# Autodesk Inventor assembly: Base Chassis Assembly
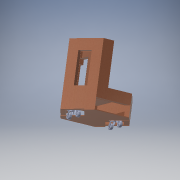
[picture p0: Inventor's stored thumbnail of the model, 180x180]
Saved by Autodesk Inventor 2017 (Build 210142000, 142)
## iProperties
Created: 2018-10-18
Part Number: Base Chassis Assembly
Document SubType Name: Assembly
Designer: Dell
Author: Dell
## Documents named in this file (13)
- C:\Users\Dell\Documents\GitHub\tr2\Base\Base Chassis Assembly.iam
- C:\Users\Dell\Documents\GitHub\tr2\BA01.ipt
- C:\Users\Dell\Documents\GitHub\tr2\BA02.ipt
- C:\Users\Dell\Documents\GitHub\tr2\Base\BA07.ipt
- C:\Users\Dell\Documents\GitHub\tr2\Base\BA08.ipt
- C:\Users\Dell\Documents\GitHub\tr2\Base\BA11.ipt
- C:\Users\Dell\Documents\GitHub\tr2\Base\BA015.ipt
- C:\Users\Dell\Documents\GitHub\tr2\Base\Caster 2in.ipt
- C:\Users\Dell\Documents\GitHub\tr2\Base\BA16.ipt
- C:\Users\Dell\Documents\GitHub\tr2\Base\BA17.ipt
- C:\Users\Dell\Documents\GitHub\tr2\Base\BA18.ipt
- C:\Users\Dell\Documents\GitHub\tr2\Base\BA22.ipt
- C:\Users\Dell\Documents\GitHub\tr2\Base\BA23.ipt
## Components (34 placed, 12 different names)
1. BA01:1
2. BA01:2 — Flush:33
3. BA01:3
4. BA01:4 — Flush:24
5. BA01:5 — Flush:32, Mate:65, Mate:67
6. BA01:6
7. BA01:7 — Mate:45, Flush:25, Mate:60
8. BA01:8 — Mate:47, Flush:26, Mate:49, Mate:55
9. BA01:9 — Mate:46, Mate:48, Mate:50, Mate:56
10. BA01:10 — Flush:24, Mate:45, Flush:25, Mate:61
11. BA02:2 — Mate:66, Mate:67, Flush:33
12. BA02:4 — Mate:64
13. BA02:5 — Flush:32, Mate:64, Mate:65, Mate:66
14. BA07:1
15. BA07:2
16. BA07:3 — Mate:76
17. BA07:4
18. BA07:5 — Mate:69, Mate:75, Flush:37
19. BA07:6 — Mate:71, Mate:74
20. BA08:1
21. BA08:2 — Mate:72
22. BA11:1 — Mate:68, Flush:34
23. BA015:1 — Mate:46, Mate:47, Mate:48
24. BA16:1 — Flush:26, Mate:49, Mate:50, Mate:51, Mate:53, Mate:54, Flush:27, Flush:29
25. BA16:2 — Mate:60, Mate:61, Flush:29, Flush:30, Flush:31
26. BA17:1 — Mate:68, Flush:34, Mate:69, Mate:70, Flush:35, Flush:36, Mate:73, Mate:77
27. BA18:1 — Mate:70, Flush:35, Mate:71
28. BA18:2 — Flush:36, Mate:72, Mate:73, Flush:38
29. Caster 2in:1 — Mate:51, Flush:27, Mate:55, Mate:63
30. Caster 2in:2 — Mate:53, Mate:54, Mate:56, Mate:62
31. Caster 2in:3 — Flush:31, Mate:63
32. Caster 2in:4 — Mate:62, Flush:30
33. BA22:1 — Mate:74, Mate:75, Flush:37
34. BA23:1 — Mate:76, Flush:38, Mate:77
## Relationships (100: Mate 68, Flush 32)
- [Mate]: BA01:1 ↔ BA01:6
- [Mate]: BA01:2 ↔ BA01:6
- [Mate]: BA01:2 ↔ BA01:6
- [Mate]: BA01:2 ↔ BA01:6
- [Flush]: BA01:1 ↔ BA01:6
- [Mate]: BA01:1 ↔ BA01:6
- [Mate]: BA01:2 ↔ BA01:3
- [Mate]: BA01:2 ↔ BA01:3
- [Flush]: BA01:2 ↔ BA01:3
- [Mate]: BA01:1 ↔ BA01:5
- [Flush]: BA01:1 ↔ BA01:5
- [Mate]: BA01:1 ↔ BA01:5
- [Mate]: BA01:4 ↔ BA01:5
- [Flush]: BA01:4 ↔ BA01:5
- [Mate]: BA01:4 ↔ BA01:5
- [Mate]: BA01:3 ↔ BA01:7
- [Mate]: BA01:3 ↔ BA01:7
- [Mate]: BA01:2 ↔ BA01:7
- [Flush]: BA01:6 ↔ BA01:8
- [Mate]: BA01:2 ↔ BA01:8
- [Mate]: BA01:6 ↔ BA01:8
- [Mate]: BA01:6 ↔ BA01:8
- [Mate]: BA01:8 ↔ BA01:9
- [Mate]: BA01:5 ↔ BA01:9
- [Mate]: BA01:1 ↔ BA01:9
- [Mate]: BA01:4 ↔ BA07:1
- [Flush]: BA01:4 ↔ BA07:1
- [Mate]: BA01:4 ↔ BA07:1
- [Mate]: BA07:1 ↔ BA07:2
- [Flush]: BA07:1 ↔ BA07:2
- [Flush]: BA01:3 ↔ BA07:2
- [Mate]: BA01:4 ↔ BA07:3
- [Flush]: BA07:1 ↔ BA07:3
- [Mate]: BA01:5 ↔ BA07:3
- [Mate]: BA07:3 ↔ BA07:4
- [Mate]: BA07:5 ↔ BA07:6
- [Mate]: BA07:5 ↔ BA07:6
- [Flush]: BA07:5 ↔ BA07:6
- [Mate]: BA01:2 ↔ BA07:6
- [Mate]: BA01:3 ↔ BA07:6
- [Flush]: BA01:7 ↔ BA07:6
- [Mate]: BA07:2 ↔ BA08:1
- [Flush]: BA07:2 ↔ BA08:1
- [Flush]: BA07:2 ↔ BA08:1
- [Mate]: BA07:1 ↔ BA08:2
- [Flush]: BA07:1 ↔ BA08:2
- [Flush]: BA07:1 ↔ BA08:2
- [Mate]: BA07:3 ↔ BA07:4
- [Mate]: BA01:5 ↔ BA07:4
- [Flush]: BA02:4 ↔ BA07:5
- [Mate]: BA02:4 ↔ BA07:4
- [Flush] (-44.45 mm): BA01:2 ↔ BA02:4
- [Mate]: BA02:4 ↔ BA11:1
- [Flush]: BA02:4 ↔ BA11:1
- [Mate] (171.45 mm): BA07:4 ↔ BA11:1
- Flush:24: BA01:4 ↔ BA01:10
- Mate:45: BA01:7 ↔ BA01:10
- Flush:25: BA01:7 ↔ BA01:10
- Mate:46: BA01:9 ↔ BA015:1
- Mate:47: BA01:8 ↔ BA015:1
- Mate:48: BA01:9 ↔ BA015:1
- Flush:26 (19.05 mm): BA01:8 ↔ BA16:1
- Mate:49: BA01:8 ↔ BA16:1
- Mate:50: BA01:9 ↔ BA16:1
- Mate:51: BA16:1 ↔ Caster 2in:1
- Mate:53: BA16:1 ↔ Caster 2in:2
- Mate:54: BA16:1 ↔ Caster 2in:2
- Flush:27: BA16:1 ↔ Caster 2in:1
- Mate:55 (12.7 mm): BA01:8 ↔ Caster 2in:1
- Mate:56 (12.7 mm): BA01:9 ↔ Caster 2in:2
- [Mate]: BA16:2 ↔ Caster 2in:3
- [Mate]: BA16:2 ↔ Caster 2in:4
- Mate:60: BA01:7 ↔ BA16:2
- Mate:61: BA01:10 ↔ BA16:2
- Flush:29: BA16:1 ↔ BA16:2
- Mate:62: Caster 2in:2 ↔ Caster 2in:4
- Flush:30: BA16:2 ↔ Caster 2in:4
- Flush:31: BA16:2 ↔ Caster 2in:3
- Mate:63: Caster 2in:1 ↔ Caster 2in:3
- Flush:32: BA01:5 ↔ BA02:5
- Mate:64: BA02:4 ↔ BA02:5
- Mate:65: BA01:5 ↔ BA02:5
- Mate:66: BA02:2 ↔ BA02:5
- Mate:67: BA01:5 ↔ BA02:2
- Flush:33: BA01:2 ↔ BA02:2
- Mate:68: BA11:1 ↔ BA17:1
- Flush:34: BA11:1 ↔ BA17:1
- Mate:69 (38.1 mm): BA07:5 ↔ BA17:1
- Mate:70: BA17:1 ↔ BA18:1
- Flush:35: BA17:1 ↔ BA18:1
- Mate:71: BA07:6 ↔ BA18:1
- Flush:36: BA17:1 ↔ BA18:2
- Mate:72: BA08:2 ↔ BA18:2
- Mate:73: BA17:1 ↔ BA18:2
- Mate:74: BA07:6 ↔ BA22:1
- Mate:75: BA07:5 ↔ BA22:1
- Flush:37 (38.1 mm): BA07:5 ↔ BA22:1
- Mate:76: BA07:3 ↔ BA23:1
- Flush:38 (38.1 mm): BA18:2 ↔ BA23:1
- Mate:77: BA17:1 ↔ BA23:1
## Named parameters: d116_d113 = 0 mm, d115_d98 = 0 mm, d122_d101 = 0 mm
